# Autodesk Inventor assembly: ASY PNS 1690 Filter legs D1000_1200
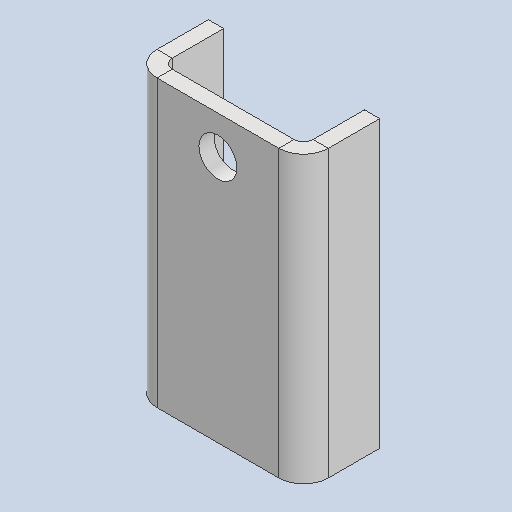
[picture p0: Inventor's stored thumbnail of the model, 512x512]
Saved by Autodesk Inventor 2026.2 (Build 302298000, 298)
## iProperties
Created: 2025-02-20
Part Number: ASY PNS 1690 Filter legs D1000_1200
Document SubType Name: Assembly
Designer: admin
Mass: 20950.1 g
Surface Area: 14148.6 cm^2
Volume: 2651.55 cm^3
Density: 7.9011 g/cm^3
Author: user
## Documents named in this file (7)
- C:\Users\admin\Documents\Inventor\PRS-Purovsk\DRS 940\ASY PNS 1690 Filter legs D1000_1200.iam
- C:\Users\admin\Documents\Inventor\PRS-Purovsk\DRS 940\PNS 1692 Leg tube.ipt
- C:\Users\admin\Documents\Inventor\PRS-Purovsk\DRS 940\PNS 1693 leg sketch_1200.ipt
- C:\Users\admin\Documents\Inventor\PRS-Purovsk\DRS 940\PNS 1694 leg plate for filter_1200.ipt
- C:\Users\admin\Documents\Inventor\PRS-Purovsk\DRS 940\PNS 1695 leg floor plate_1200.ipt
- C:\Users\admin\Documents\Inventor\PRS-Purovsk\DRS 940\PNS 1785 leg floor channel_1200.ipt
- C:\Users\admin\Documents\Inventor\PRS-Purovsk\DRS 940\PNS 1696 leg floor pattern.ipt
## Components (6 placed, 6 different names)
1. PNS 1692 Leg tube:1 — Mate:4, Mate:6, Mate:7, Flush:1, Mate:5
2. PNS 1693 leg sketch_1200:1 — Mate:6
3. PNS 1694 leg plate for filter_1200:1 — Mate:7
4. PNS 1695 leg floor plate_1200:1 — Flush:1, Mate:5, Rigid:10
5. PNS 1785 leg floor channel_1200:1 — Mate:2, Mate:1, Rigid:10
6. PNS 1696 leg floor pattern:1
## Relationships (8: Mate 6, Flush 1, WeldJoint 1)
- Mate:4: PNS 1692 Leg tube:1
- Mate:6: PNS 1692 Leg tube:1 ↔ PNS 1693 leg sketch_1200:1
- Mate:7: PNS 1692 Leg tube:1 ↔ PNS 1694 leg plate for filter_1200:1
- Flush:1 (5 mm): PNS 1692 Leg tube:1 ↔ PNS 1695 leg floor plate_1200:1
- Mate:5: PNS 1692 Leg tube:1 ↔ PNS 1695 leg floor plate_1200:1
- Mate:2: PNS 1785 leg floor channel_1200:1
- Mate:1: PNS 1785 leg floor channel_1200:1
- Rigid:10 [WeldJoint]: PNS 1695 leg floor plate_1200:1 ↔ PNS 1785 leg floor channel_1200:1
## Named parameters: Out_diam = 963 mm
